# Autodesk Inventor assembly: Evo
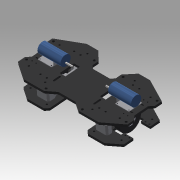
[picture p0: Inventor's stored thumbnail of the model, 180x180]
Saved by Autodesk Inventor 2016 (Build 200138000, 138)
## iProperties
Created: 2017-12-05
Part Number: Evo
Material: Générique
Document SubType Name: Assembly
Designer: LogOut
Author: LogOut
## Documents named in this file (6)
- C:\Travail\Objets\GitHub\Evo_Mechanical\Mechanic\Modelisation\Evo.iam
- C:\Travail\Objets\GitHub\Evo_Mechanical\Mechanic\Modelisation\Wheel_Support.ipt
- C:\Travail\Objets\GitHub\Evo_Mechanical\Mechanic\Modelisation\Motor_Support.ipt
- C:\Travail\Objets\GitHub\Evo_Mechanical\Mechanic\Modelisation\Wheel_Block.ipt
- C:\Travail\Objets\GitHub\Evo_Mechanical\Mechanic\Modelisation\Motor.ipt
- C:\Travail\Objets\GitHub\Evo_Mechanical\Mechanic\Modelisation\Motor_Wheel.ipt
## Components (9 placed, 5 different names)
1. Motor_Support:1 — Placage:1, Placage:3, Placage:4, Placage:5, Placage:6, Placage:7, Placage:8, Placage:9, Placage:10, Placage:11, Placage:12, Placage:13, Placage:14, Placage:15
2. Wheel_Support:1 — Placage:3, Placage:8, Affleurement:1, Placage:17
3. Wheel_Support:2 — Placage:1, Placage:9, Affleurement:1, Placage:19
4. Wheel_Block:1 — Placage:4, Placage:6, Affleurement:2, Placage:16
5. Wheel_Block:2 — Placage:5, Placage:7, Affleurement:2, Placage:18
6. Motor:1 — Placage:10, Placage:11, Placage:12
7. Motor:2 — Placage:13, Placage:14, Placage:15
8. Motor_Wheel:1 — Placage:16, Placage:17
9. Motor_Wheel:2 — Placage:18, Placage:19
## Relationships (20: Mate 18, Flush 2)
- Placage:1 [Mate]: Motor_Support:1 ↔ Wheel_Support:2
- Placage:3 [Mate]: Motor_Support:1 ↔ Wheel_Support:1
- Placage:4 [Mate]: Motor_Support:1 ↔ Wheel_Block:1
- Placage:5 [Mate]: Motor_Support:1 ↔ Wheel_Block:2
- Placage:6 [Mate]: Motor_Support:1 ↔ Wheel_Block:1
- Placage:7 [Mate]: Motor_Support:1 ↔ Wheel_Block:2
- Placage:8 [Mate]: Motor_Support:1 ↔ Wheel_Support:1
- Placage:9 [Mate]: Motor_Support:1 ↔ Wheel_Support:2
- Affleurement:1 [Flush]: Wheel_Support:1 ↔ Wheel_Support:2
- Affleurement:2 [Flush]: Wheel_Block:1 ↔ Wheel_Block:2
- Placage:10 [Mate]: Motor_Support:1 ↔ Motor:1
- Placage:11 [Mate]: Motor_Support:1 ↔ Motor:1
- Placage:12 [Mate]: Motor_Support:1 ↔ Motor:1
- Placage:13 [Mate]: Motor_Support:1 ↔ Motor:2
- Placage:14 [Mate]: Motor_Support:1 ↔ Motor:2
- Placage:15 [Mate]: Motor_Support:1 ↔ Motor:2
- Placage:16 [Mate]: Wheel_Block:1 ↔ Motor_Wheel:1
- Placage:17 [Mate] (4 mm): Wheel_Support:1 ↔ Motor_Wheel:1
- Placage:18 [Mate]: Wheel_Block:2 ↔ Motor_Wheel:2
- Placage:19 [Mate] (4 mm): Wheel_Support:2 ↔ Motor_Wheel:2
